# Autodesk Inventor assembly: subassembly_auger_case
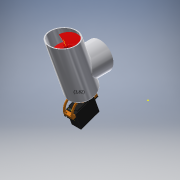
[picture p0: Inventor's stored thumbnail of the model, 180x180]
Saved by Autodesk Inventor 2019 (Build 230136000, 136)
## iProperties
Created: 2019-01-23
Part Number: subassembly_auger_case
Document SubType Name: Assembly
Designer: jmc
Author: jmc
## Documents named in this file (6)
- C:\Users\l0086\Desktop\Models\CatFeeder\version4 (auger)\subassembly_auger_case.iam
- C:\Users\l0086\Desktop\Models\CatFeeder\Auger\auger.ipt
- C:\Users\l0086\Desktop\Models\CatFeeder\Auger\screw.ipt
- C:\Users\l0086\Desktop\Models\3party\Servos\MG995.ipt
- C:\Users\l0086\Desktop\Models\CatFeeder\Auger\servo_adapter.ipt
- C:\Users\l0086\Desktop\Models\CatFeeder\Auger\servo_holder.ipt
## Components (5 placed, 5 different names)
1. auger:1 — Rotational:1, Rigid:3
2. screw:1 — Rotational:1, Rigid:1
3. MG995:1 — Rigid:4
4. servo_adapter:1 — Rigid:1
5. servo_holder:1 — Rigid:3, Rigid:4
## Relationships (4: WeldJoint 3, RevoluteJoint 1)
- Rotational:1 [RevoluteJoint]: auger:1 ↔ screw:1
- Rigid:1 [WeldJoint]: screw:1 ↔ servo_adapter:1
- Rigid:3 [WeldJoint]: auger:1 ↔ servo_holder:1
- Rigid:4 [WeldJoint]: MG995:1 ↔ servo_holder:1
